# Autodesk Inventor assembly: IMUSupportAssembly
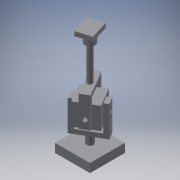
[picture p0: Inventor's stored thumbnail of the model, 180x180]
Saved by Autodesk Inventor 2016 (Build 200138000, 138)
## iProperties
Created: 2017-04-12
Part Number: IMUSupportAssembly
Document SubType Name: Assembly
Designer: Evan Phil George
Author: Evan Phil George
## Documents named in this file (6)
- C:\Users\Evan Phil George\Desktop\Ball Balancing Robot\TestBenchInventor\OpticalSensorSupport\IMUSupportAssembly.iam
- C:\Users\Evan Phil George\Desktop\Ball Balancing Robot\TestBenchInventor\OpticalSensorSupport\Base.ipt
- C:\Users\Evan Phil George\Desktop\Ball Balancing Robot\TestBenchInventor\OpticalSensorSupport\BaseFork.ipt
- C:\Users\Evan Phil George\Desktop\Ball Balancing Robot\TestBenchInventor\OpticalSensorSupport\TopFork.ipt
- C:\Users\Evan Phil George\Desktop\Ball Balancing Robot\TestBenchInventor\OpticalSensorSupport\coupling.ipt
- C:\Users\Evan Phil George\Desktop\Ball Balancing Robot\TestBenchInventor\OpticalSensorSupport\imusupport.ipt
## Components (5 placed, 5 different names)
1. Base:1 — Mate:3, Mate:4, Angle:1
2. BaseFork:1 — Mate:3, Mate:4, Mate:5, Mate:6
3. TopFork:1 — Mate:1, Mate:2, Mate:7, Mate:8
4. coupling:1 — Mate:5, Mate:6, Mate:7, Mate:8
5. imusupport:1 — Mate:1, Mate:2, Angle:1
## Relationships (9: Mate 8, Angle 1)
- Mate:1: TopFork:1 ↔ imusupport:1
- Mate:2: TopFork:1 ↔ imusupport:1
- Mate:3: Base:1 ↔ BaseFork:1
- Mate:4: Base:1 ↔ BaseFork:1
- Mate:5: BaseFork:1 ↔ coupling:1
- Mate:6: BaseFork:1 ↔ coupling:1
- Mate:7: TopFork:1 ↔ coupling:1
- Mate:8: TopFork:1 ↔ coupling:1
- Angle:1 (0 deg): Base:1 ↔ imusupport:1
